# Autodesk Inventor assembly: Grab mount
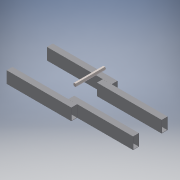
[picture p0: Inventor's stored thumbnail of the model, 180x180]
Saved by Autodesk Inventor 2019 (Build 230136000, 136)
## iProperties
Created: 2019-02-04
Part Number: Grab mount
Document SubType Name: Assembly
Designer: josh
Author: josh
## Documents named in this file (3)
- D:\Synthesis Robots\Epsilon\Epsilon Grabbers\Grabbing unit\Grab mount.iam
- D:\Synthesis Robots\Epsilon\Epsilon Grabbers\Aluminum grabber mount.ipt
- D:\Synthesis Robots\Epsilon\Epsilon Grabbers\Bag Motor parts\am-0856 500 Hex Shaft for Modulox REV3.ipt
## Components (5 placed, 2 different names)
1. Aluminum grabber mount:1 — Flush:1, Flush:2, Mate:1, Flush:3, Mate:2
2. Aluminum grabber mount:2 — Flush:1, Flush:2, Flush:4, Mate:3, Mate:4
3. Aluminum grabber mount:3 — Mate:1, Flush:3, Mate:2
4. Aluminum grabber mount:4 — Flush:4, Mate:3, Mate:4
5. am-0856 500 Hex Shaft for Modulox REV3:1
## Relationships (8: Flush 4, Mate 4)
- Flush:1: Aluminum grabber mount:1 ↔ Aluminum grabber mount:2
- Flush:2: Aluminum grabber mount:1 ↔ Aluminum grabber mount:2
- Mate:1: Aluminum grabber mount:1 ↔ Aluminum grabber mount:3
- Flush:3: Aluminum grabber mount:1 ↔ Aluminum grabber mount:3
- Mate:2 (-38.1 mm): Aluminum grabber mount:1 ↔ Aluminum grabber mount:3
- Flush:4: Aluminum grabber mount:2 ↔ Aluminum grabber mount:4
- Mate:3: Aluminum grabber mount:2 ↔ Aluminum grabber mount:4
- Mate:4 (-38.1 mm): Aluminum grabber mount:2 ↔ Aluminum grabber mount:4
